# Autodesk Inventor assembly: Assembly3
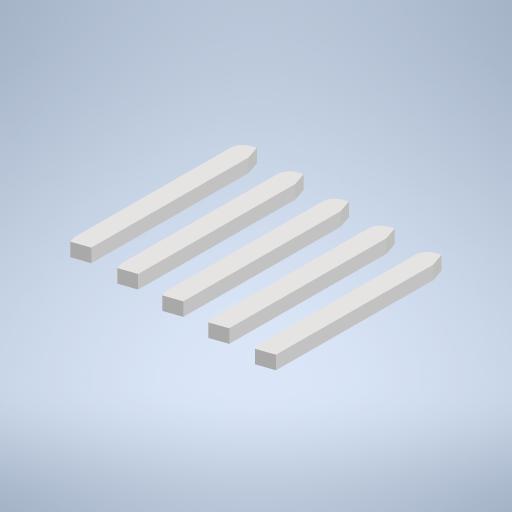
[picture p0: Inventor's stored thumbnail of the model, 512x512]
Saved by Autodesk Inventor 2023.1 (Build 271208000, 208)
## iProperties
Created: 2022-11-04
Part Number: Assembly3
Document SubType Name: Assembly
Designer: jshin23
Author: jshin23
## Documents named in this file (2)
- C:\Users\jshin23\Desktop\Kids Toy\Assembly3.iam
- C:\Users\jshin23\Desktop\Kids Toy\Part4 x 12.ipt
## Components (5 placed, 1 different names)
1. Part4 x 12:1 — Flush:1, Flush:4, Mate:1, Mate:2
2. Part4 x 12:2 — Flush:1, Flush:2, Flush:3, Mate:2, Mate:5
3. Part4 x 12:3 — Flush:2, Mate:4
4. Part4 x 12:4 — Flush:4, Mate:4, Mate:5
5. Part4 x 12:5 — Flush:3, Mate:1
## Relationships (8: Flush 4, Mate 4)
- Flush:1: Part4 x 12:1 ↔ Part4 x 12:2
- Flush:2: Part4 x 12:2 ↔ Part4 x 12:3
- Flush:3: Part4 x 12:2 ↔ Part4 x 12:5
- Flush:4: Part4 x 12:1 ↔ Part4 x 12:4
- Mate:1 (20.32 mm): Part4 x 12:1 ↔ Part4 x 12:5
- Mate:2 (20.32 mm): Part4 x 12:1 ↔ Part4 x 12:2
- Mate:4 (20.32 mm): Part4 x 12:3 ↔ Part4 x 12:4
- Mate:5 (20.32 mm): Part4 x 12:2 ↔ Part4 x 12:4
